# Autodesk Inventor assembly: DriveMotorAssem
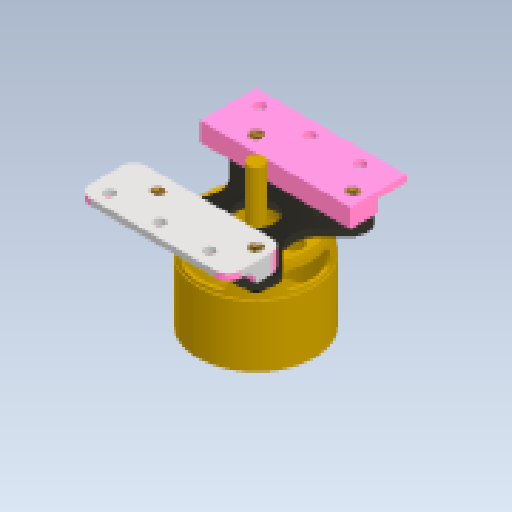
[picture p0: Inventor's stored thumbnail of the model, 512x512]
Saved by Autodesk Inventor 2023 (Build 270158000, 158)
## iProperties
Created: 2023-03-30
Part Number: DriveMotorAssem
Document SubType Name: Assembly
Designer: Dave
Mass: 268.152 g
Surface Area: 522.44 cm^2
Volume: 82.9291 cm^3
Density: 3.2335 g/cm^3
Author: Dave
## Documents named in this file (7)
- C:\Users\Dave\Documents\GitHub\BehrendURCMechanical\CAD\Chassis V3\DriveMotorAssem\DriveMotorAssem.iam
- C:\Users\Dave\Documents\GitHub\BehrendURCMechanical\CAD\Chassis V3\DriveMotorPlate.ipt
- C:\Users\Dave\Documents\GitHub\BehrendURCMechanical\CAD\Chassis V3\DriveMotorAssem\Drive Motor.ipt
- C:\Users\Dave\Downloads\91290A148_Alloy Steel Socket Head Screw.ipt
- C:\Users\Dave\Downloads\94180A351_Tapered Heat-Set Inserts for Plastic.ipt
- C:\Users\Dave\Documents\GitHub\BehrendURCMechanical\CAD\Chassis V3\DriveMotorAssem\DriveMotorMount5.ipt
- C:\Users\Dave\Documents\GitHub\BehrendURCMechanical\CAD\Chassis V3\DriveMotorAssem\DriveMotorMount5_MIR1.ipt
## Components (12 placed, 6 different names)
1. DriveMotorPlate:1 — Insert:1, Insert:2, Insert:9, Insert:10, Insert:11, Insert:12, Insert:13, Insert:17, Insert:18
2. Drive Motor:1 — Insert:1, Insert:2
3. 91290A148_Alloy Steel Socket Head Screw:1 — Insert:9
4. 94180A351_Tapered Heat-Set Inserts for Plastic:1 — Insert:20
5. 91290A148_Alloy Steel Socket Head Screw:2 — Insert:10, Mate:1
6. 94180A351_Tapered Heat-Set Inserts for Plastic:2 — Insert:19
7. 91290A148_Alloy Steel Socket Head Screw:3 — Insert:11
8. 94180A351_Tapered Heat-Set Inserts for Plastic:3 — Insert:16
9. 91290A148_Alloy Steel Socket Head Screw:4 — Insert:12
10. 94180A351_Tapered Heat-Set Inserts for Plastic:4 — Insert:15
11. DriveMotorMount5:2 — Insert:13, Mate:1, Insert:15, Insert:16
12. DriveMotorMount5_MIR1:1 — Insert:17, Insert:18, Insert:19, Insert:20
## Relationships (14: Insert 13, Mate 1)
- Insert:1: DriveMotorPlate:1 ↔ Drive Motor:1
- Insert:2: DriveMotorPlate:1 ↔ Drive Motor:1
- Insert:9: DriveMotorPlate:1 ↔ 91290A148_Alloy Steel Socket Head Screw:1
- Insert:10: DriveMotorPlate:1 ↔ 91290A148_Alloy Steel Socket Head Screw:2
- Insert:11: DriveMotorPlate:1 ↔ 91290A148_Alloy Steel Socket Head Screw:3
- Insert:12: DriveMotorPlate:1 ↔ 91290A148_Alloy Steel Socket Head Screw:4
- Insert:13: DriveMotorPlate:1 ↔ DriveMotorMount5:2
- Mate:1: 91290A148_Alloy Steel Socket Head Screw:2 ↔ DriveMotorMount5:2
- Insert:15: 94180A351_Tapered Heat-Set Inserts for Plastic:4 ↔ DriveMotorMount5:2
- Insert:16: 94180A351_Tapered Heat-Set Inserts for Plastic:3 ↔ DriveMotorMount5:2
- Insert:17: DriveMotorPlate:1 ↔ DriveMotorMount5_MIR1:1
- Insert:18: DriveMotorPlate:1 ↔ DriveMotorMount5_MIR1:1
- Insert:19: 94180A351_Tapered Heat-Set Inserts for Plastic:2 ↔ DriveMotorMount5_MIR1:1
- Insert:20: 94180A351_Tapered Heat-Set Inserts for Plastic:1 ↔ DriveMotorMount5_MIR1:1
